# Autodesk Inventor assembly: mount
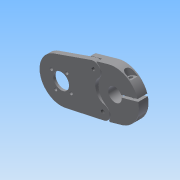
[picture p0: Inventor's stored thumbnail of the model, 180x180]
Saved by Autodesk Inventor 2015 (Build 190159000, 159)
## iProperties
Created: 2014-11-17
Part Number: mount
Document SubType Name: Assembly
Designer: brent
Author: brent
## Documents named in this file (9)
- C:\Users\brent\Documents\electric-longboard\brent2\mount.iam
- C:\Users\brent\Documents\electric-longboard\brent2\mount_base.ipt
- C:\Users\brent\Documents\electric-longboard\brent2\mount_plate.ipt
- C:\Users\brent\Documents\electric-longboard\brent2\mount\AIP\FEA\b8n8xrom8.fins
- C:\Users\brent\Documents\electric-longboard\brent2\mount\AIP\FEA\b8n8xrom8.fsat
- C:\Users\brent\Documents\electric-longboard\brent2\mount\AIP\FEA\b8n8xrom8.ftes
- C:\Users\brent\Documents\electric-longboard\brent2\mount\AIP\FEA\b8n8xrom8.fwiz
- C:\Users\brent\Documents\electric-longboard\brent2\mount\AIP\FEA\b8n8xrou8.fmsh
- C:\Users\brent\Documents\electric-longboard\brent2\mount\AIP\FEA\b8n8xrou9.fres
## Components (2 placed, 2 different names)
1. mount_base:1 — Mate:1, Mate:2, Mate:3
2. mount_plate:1 — Mate:1, Mate:2, Mate:3
## Relationships (3: Mate 3)
- Mate:1: mount_base:1 ↔ mount_plate:1
- Mate:2: mount_base:1 ↔ mount_plate:1
- Mate:3: mount_base:1 ↔ mount_plate:1
## Named parameters: sa_0 = -1.33447e-11, sa_1 = 4.44822e-12, sa_2 = 44482.2, sa_3 = 24095.2, sa_4 = -85639.3, sa_5 = -0, sa_6 = -24095.2, sa_7 = 85639.3, sa_8 = -0
note: some values were not read from the file. Shown as the stored number, unit unknown: "sa_0", "sa_1", "sa_2", "sa_3", "sa_4", "sa_5", "sa_6", "sa_7", "sa_8".
